# Autodesk Inventor assembly: Y-Carriage_LM3037_v2
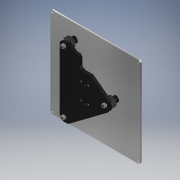
[picture p0: Inventor's stored thumbnail of the model, 180x180]
Saved by Autodesk Inventor 2020.3 (Build 243373000, 373)
## iProperties
Created: 2020-05-30
Part Number: Y-Carriage_LM3037_v2
Document SubType Name: Assembly
Designer: rah75
Author: rah75
## Documents named in this file (11)
- C:\Users\rah75\Documents\GitHub\LETU-Maker\CAD\Autodesk Inventor\Base_3001-5999\Y-Carriage\Assemblies\Y-Carriage_Low_Profile_LM3050.iam
- C:\Users\rah75\Documents\GitHub\LETU-Maker\CAD\Autodesk Inventor\Stock_Components_1001-2999\Power_Transmission\Bearings\V-Groove_Bearing_5mm_LM1041.ipt
- C:\Users\rah75\Documents\GitHub\LETU-Maker\CAD\Autodesk Inventor\Base_3001-5999\Y-Carriage\Fabricated_Parts\Y-Carriage_Lower_Plate_LM3039.ipt
- C:\Users\rah75\Documents\GitHub\LETU-Maker\CAD\Autodesk Inventor\Base_3001-5999\Y-Carriage\Fabricated_Parts\Y-Carriage_Plate_LM3033_v2.ipt
- C:\Users\rah75\Documents\GitHub\LETU-Maker\CAD\Autodesk Inventor\Base_3001-5999\Y-Carriage\Printed_Parts\Y-Carraige_Spacer_LM3044.ipt
- C:\Users\rah75\Documents\GitHub\LETU-Maker\CAD\Autodesk Inventor\Base_3001-5999\X-Carriage\Printed_Parts\X-Carriage_Belt_Clamp_LM3007.ipt
- C:\Users\rah75\Documents\GitHub\LETU-Maker\CAD\Autodesk Inventor\Stock_Components_1001-2999\Fasteners\Washers_Spacers\washer_m5_LM1002.ipt
- C:\Users\rah75\Documents\GitHub\LETU-Maker\CAD\Autodesk Inventor\Stock_Components_1001-2999\Fasteners\Screws\BHHD_m5x35_LM1050.ipt
- C:\Users\rah75\Documents\GitHub\LETU-Maker\CAD\Autodesk Inventor\Stock_Components_1001-2999\Fasteners\Nuts\hex_nut_m5_LM1020.ipt
- C:\Users\rah75\Documents\GitHub\LETU-Maker\CAD\Autodesk Inventor\Stock_Components_1001-2999\Fasteners\Nuts\heat_insert_m3_LM1017.ipt
- C:\Users\rah75\Documents\GitHub\LETU-Maker\CAD\Autodesk Inventor\Stock_Components_1001-2999\Fasteners\Screws\SHCS_m3x8_LM1008.ipt
## Components (30 placed, 10 different names)
1. V-Groove_Bearing_5mm_LM1041:1 — Flush:5, Mate:7, Mate:8, Mate:9, Mate:20, Insert:16, Insert:22
2. V-Groove_Bearing_5mm_LM1041:2 — Flush:4, Mate:7, Mate:9, Insert:14, Insert:17, Insert:23
3. V-Groove_Bearing_5mm_LM1041:3 — Flush:4, Flush:5, Mate:8, Insert:15, Insert:24
4. Y-Carriage_Lower_Plate_LM3039:1 — Insert:20, Insert:21, Mate:21, Mate:22, Insert:25, Mate:23, Insert:30, Insert:31, Insert:32, Insert:36, Insert:37, Insert:38, Insert:39
5. Y-Carriage_Plate_LM3033_v2:1 — Insert:14, Mate:20, Insert:26, Insert:27, Insert:28, Insert:29
6. Y-Carraige_Spacer_LM3044:1 — Insert:16
7. Y-Carraige_Spacer_LM3044:2 — Insert:17, Mate:23
8. Y-Carraige_Spacer_LM3044:3 — Insert:15, Insert:26
9. X-Carriage_Belt_Clamp_LM3007:1 — Insert:20, Mate:21, Insert:40, Insert:41
10. X-Carriage_Belt_Clamp_LM3007:2 — Insert:21, Mate:22, Insert:42, Insert:43
11. washer_m5_LM1002:1 — Insert:24, Insert:25
12. washer_m5_LM1002:2 — Insert:23
13. washer_m5_LM1002:3 — Insert:22
14. BHHD_m5x35_LM1050:1 — Insert:28
15. BHHD_m5x35_LM1050:2 — Insert:29
16. BHHD_m5x35_LM1050:3 — Insert:27
17. washer_m5_LM1002:4 — Insert:30, Insert:33
18. washer_m5_LM1002:5 — Insert:31, Insert:34
19. washer_m5_LM1002:6 — Insert:32, Insert:35
20. hex_nut_m5_LM1020:1 — Insert:33
21. hex_nut_m5_LM1020:2 — Insert:34
22. hex_nut_m5_LM1020:3 — Insert:35
23. heat_insert_m3_LM1017:1 — Insert:36
24. heat_insert_m3_LM1017:2 — Insert:37
25. heat_insert_m3_LM1017:3 — Insert:38
26. heat_insert_m3_LM1017:4 — Insert:39
27. SHCS_m3x8_LM1008:1 — Insert:40
28. SHCS_m3x8_LM1008:2 — Insert:41
29. SHCS_m3x8_LM1008:3 — Insert:42
30. SHCS_m3x8_LM1008:4 — Insert:43
## Relationships (37: Insert 28, Mate 7, Flush 2)
- Flush:4: V-Groove_Bearing_5mm_LM1041:2 ↔ V-Groove_Bearing_5mm_LM1041:3
- Flush:5: V-Groove_Bearing_5mm_LM1041:1 ↔ V-Groove_Bearing_5mm_LM1041:3
- Mate:7 (75 mm): V-Groove_Bearing_5mm_LM1041:1 ↔ V-Groove_Bearing_5mm_LM1041:2
- Mate:8 (150 mm): V-Groove_Bearing_5mm_LM1041:1 ↔ V-Groove_Bearing_5mm_LM1041:3
- Mate:9 (75 mm): V-Groove_Bearing_5mm_LM1041:1 ↔ V-Groove_Bearing_5mm_LM1041:2
- Insert:14 (8 mm): V-Groove_Bearing_5mm_LM1041:2 ↔ Y-Carriage_Plate_LM3033_v2:1
- Mate:20: V-Groove_Bearing_5mm_LM1041:1 ↔ Y-Carriage_Plate_LM3033_v2:1
- Insert:15: V-Groove_Bearing_5mm_LM1041:3 ↔ Y-Carraige_Spacer_LM3044:3
- Insert:16: V-Groove_Bearing_5mm_LM1041:1 ↔ Y-Carraige_Spacer_LM3044:1
- Insert:17: V-Groove_Bearing_5mm_LM1041:2 ↔ Y-Carraige_Spacer_LM3044:2
- Insert:20: Y-Carriage_Lower_Plate_LM3039:1 ↔ X-Carriage_Belt_Clamp_LM3007:1
- Insert:21: Y-Carriage_Lower_Plate_LM3039:1 ↔ X-Carriage_Belt_Clamp_LM3007:2
- Mate:21: Y-Carriage_Lower_Plate_LM3039:1 ↔ X-Carriage_Belt_Clamp_LM3007:1
- Mate:22: Y-Carriage_Lower_Plate_LM3039:1 ↔ X-Carriage_Belt_Clamp_LM3007:2
- Insert:22: V-Groove_Bearing_5mm_LM1041:1 ↔ washer_m5_LM1002:3
- Insert:23: V-Groove_Bearing_5mm_LM1041:2 ↔ washer_m5_LM1002:2
- Insert:24: V-Groove_Bearing_5mm_LM1041:3 ↔ washer_m5_LM1002:1
- Insert:25: Y-Carriage_Lower_Plate_LM3039:1 ↔ washer_m5_LM1002:1
- Insert:26: Y-Carriage_Plate_LM3033_v2:1 ↔ Y-Carraige_Spacer_LM3044:3
- Mate:23: Y-Carriage_Lower_Plate_LM3039:1 ↔ Y-Carraige_Spacer_LM3044:2
- Insert:27: Y-Carriage_Plate_LM3033_v2:1 ↔ BHHD_m5x35_LM1050:3
- Insert:28: Y-Carriage_Plate_LM3033_v2:1 ↔ BHHD_m5x35_LM1050:1
- Insert:29: Y-Carriage_Plate_LM3033_v2:1 ↔ BHHD_m5x35_LM1050:2
- Insert:30: Y-Carriage_Lower_Plate_LM3039:1 ↔ washer_m5_LM1002:4
- Insert:31: Y-Carriage_Lower_Plate_LM3039:1 ↔ washer_m5_LM1002:5
- Insert:32: Y-Carriage_Lower_Plate_LM3039:1 ↔ washer_m5_LM1002:6
- Insert:33: washer_m5_LM1002:4 ↔ hex_nut_m5_LM1020:1
- Insert:34: washer_m5_LM1002:5 ↔ hex_nut_m5_LM1020:2
- Insert:35: washer_m5_LM1002:6 ↔ hex_nut_m5_LM1020:3
- Insert:36: Y-Carriage_Lower_Plate_LM3039:1 ↔ heat_insert_m3_LM1017:1
- Insert:37: Y-Carriage_Lower_Plate_LM3039:1 ↔ heat_insert_m3_LM1017:2
- Insert:38: Y-Carriage_Lower_Plate_LM3039:1 ↔ heat_insert_m3_LM1017:3
- Insert:39: Y-Carriage_Lower_Plate_LM3039:1 ↔ heat_insert_m3_LM1017:4
- Insert:40: X-Carriage_Belt_Clamp_LM3007:1 ↔ SHCS_m3x8_LM1008:1
- Insert:41: X-Carriage_Belt_Clamp_LM3007:1 ↔ SHCS_m3x8_LM1008:2
- Insert:42: X-Carriage_Belt_Clamp_LM3007:2 ↔ SHCS_m3x8_LM1008:3
- Insert:43: X-Carriage_Belt_Clamp_LM3007:2 ↔ SHCS_m3x8_LM1008:4
